# Autodesk Inventor assembly: RhinoTrackRobotWithRevRoboticsLift
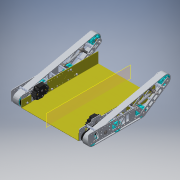
[picture p0: Inventor's stored thumbnail of the model, 180x180]
Saved by Autodesk Inventor 2019 (Build 230136000, 136)
## iProperties
Created: 2018-07-04
Part Number: RhinoTrackRobotWithRevRoboticsLift
Document SubType Name: Assembly
Designer: steele
Author: steele
## Documents named in this file (4)
- C:\git\CAD-Development\robSteele\2018PostSeasonLift\RhinoTrackRobotWithRevRoboticsLift.iam
- C:\git\CAD-Development\robSteele\2018PostSeasonLift\SheetBottomFloor.ipt
- C:\git\CAD-MfgResources\Andy-Mark\RhinoTrack\rightModules\am-3322_Rhino_Track_Drive_Module_Right.iam
- C:\git\CAD-MfgResources\Andy-Mark\RhinoTrack\leftModule\am-3322_Rhino_Track_Drive_Module_Left.iam
## Components (3 placed, 3 different names)
1. SheetBottomFloor:1 — Insert:1, Insert:2, Insert:3, Insert:4
2. am-3322_Rhino_Track_Drive_Module_Right:1 [sub-assembly] — Insert:3, Insert:4
3. am-3322_Rhino_Track_Drive_Module_Left:1 [sub-assembly] — Insert:1, Insert:2
## Relationships (4: Insert 4)
- Insert:1: SheetBottomFloor:1 ↔ am-3322_Rhino_Track_Drive_Module_Left:1
- Insert:2: SheetBottomFloor:1 ↔ am-3322_Rhino_Track_Drive_Module_Left:1
- Insert:3: SheetBottomFloor:1 ↔ am-3322_Rhino_Track_Drive_Module_Right:1
- Insert:4: SheetBottomFloor:1 ↔ am-3322_Rhino_Track_Drive_Module_Right:1
